# Autodesk Inventor assembly: assembly of dome with corridors with all doors
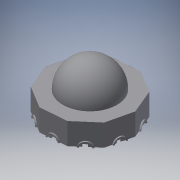
[picture p0: Inventor's stored thumbnail of the model, 180x180]
Saved by Autodesk Inventor 2017 (Build 210142000, 142)
## iProperties
Created: 2018-04-11
Part Number: assembly of dome with corridors with all doors
Document SubType Name: Assembly
Designer: Braxton
Author: Braxton
## Documents named in this file (3)
- E:\School\Game develpment\geoscape\rooms\assembly of dome with corridors with all doors.iam
- E:\School\Game develpment\geoscape\rooms\dome with corridors.ipt
- E:\School\Game develpment\geoscape\done\doors\double door.ipt
## Components (21 placed, 2 different names)
1. dome with corridors:1 — Mate:1, Mate:2, Mate:3, Mate:4, Mate:5, Mate:6, Mate:7, Mate:8, Mate:9, Mate:10, Mate:11, Mate:12, Mate:13, Mate:14, Mate:15, Mate:16, Mate:17, Mate:18, Mate:19, Mate:20, Mate:21, Mate:22, Mate:23, Mate:24, Mate:25, Mate:26, Mate:27, Mate:28, Mate:29, Mate:30, Mate:31, Mate:32, Mate:33, Mate:34, Mate:35, Mate:36, Mate:37, Mate:38, Mate:39, Mate:40
2. double door:1 — Mate:6, Mate:28
3. double door:2 — Mate:5, Mate:27
4. double door:3 — Mate:4, Mate:26
5. double door:4 — Mate:3, Mate:25
6. double door:5 — Mate:2, Mate:24
7. double door:6 — Mate:1, Mate:23
8. double door:7 — Mate:20, Mate:22
9. double door:8 — Mate:19, Mate:21
10. double door:9 — Mate:18, Mate:40
11. double door:10 — Mate:17, Mate:39
12. double door:11 — Mate:16, Mate:38
13. double door:12 — Mate:15, Mate:37
14. double door:13 — Mate:14, Mate:36
15. double door:14 — Mate:13, Mate:35
16. double door:15 — Mate:12, Mate:34
17. double door:16 — Mate:11, Mate:33
18. double door:17 — Mate:10, Mate:32
19. double door:18 — Mate:9, Mate:31
20. double door:19 — Mate:8, Mate:30
21. double door:20 — Mate:7, Mate:29
## Relationships (40: Mate 40)
- Mate:1: dome with corridors:1 ↔ double door:6
- Mate:2: dome with corridors:1 ↔ double door:5
- Mate:3: dome with corridors:1 ↔ double door:4
- Mate:4: dome with corridors:1 ↔ double door:3
- Mate:5: dome with corridors:1 ↔ double door:2
- Mate:6: dome with corridors:1 ↔ double door:1
- Mate:7: dome with corridors:1 ↔ double door:20
- Mate:8: dome with corridors:1 ↔ double door:19
- Mate:9: dome with corridors:1 ↔ double door:18
- Mate:10: dome with corridors:1 ↔ double door:17
- Mate:11: dome with corridors:1 ↔ double door:16
- Mate:12: dome with corridors:1 ↔ double door:15
- Mate:13: dome with corridors:1 ↔ double door:14
- Mate:14: dome with corridors:1 ↔ double door:13
- Mate:15: dome with corridors:1 ↔ double door:12
- Mate:16: dome with corridors:1 ↔ double door:11
- Mate:17: dome with corridors:1 ↔ double door:10
- Mate:18: dome with corridors:1 ↔ double door:9
- Mate:19: dome with corridors:1 ↔ double door:8
- Mate:20: dome with corridors:1 ↔ double door:7
- Mate:21: dome with corridors:1 ↔ double door:8
- Mate:22: dome with corridors:1 ↔ double door:7
- Mate:23: dome with corridors:1 ↔ double door:6
- Mate:24: dome with corridors:1 ↔ double door:5
- Mate:25: dome with corridors:1 ↔ double door:4
- Mate:26: dome with corridors:1 ↔ double door:3
- Mate:27: dome with corridors:1 ↔ double door:2
- Mate:28: dome with corridors:1 ↔ double door:1
- Mate:29: dome with corridors:1 ↔ double door:20
- Mate:30: dome with corridors:1 ↔ double door:19
- Mate:31: dome with corridors:1 ↔ double door:18
- Mate:32: dome with corridors:1 ↔ double door:17
- Mate:33: dome with corridors:1 ↔ double door:16
- Mate:34: dome with corridors:1 ↔ double door:15
- Mate:35: dome with corridors:1 ↔ double door:14
- Mate:36: dome with corridors:1 ↔ double door:13
- Mate:37: dome with corridors:1 ↔ double door:12
- Mate:38: dome with corridors:1 ↔ double door:11
- Mate:39: dome with corridors:1 ↔ double door:10
- Mate:40: dome with corridors:1 ↔ double door:9
